# Autodesk Inventor assembly: X Axis
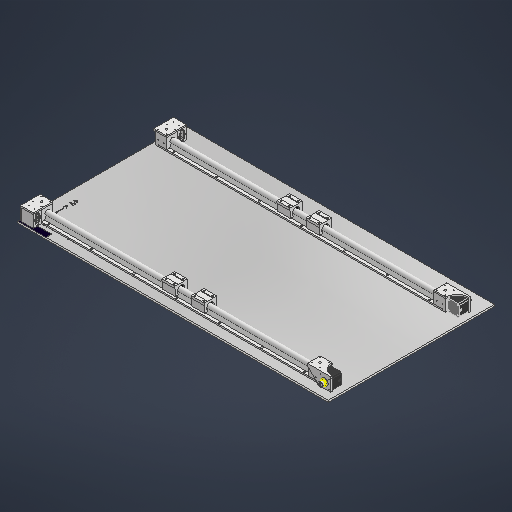
[picture p0: Inventor's stored thumbnail of the model, 512x512]
Saved by Autodesk Inventor 2025.1 (Build 291241000, 241)
## iProperties
Created: 2024-11-25
Part Number: X Axis
Document SubType Name: Assembly
Designer: jerem
Author: jerem
## Documents named in this file (8)
- C:\Users\jerem\Documents\GitHub\Perovskite-Automated-Synthesis-System\CAD\Gantry\X Axis.iam
- C:\Users\jerem\Documents\GitHub\Perovskite-Automated-Synthesis-System\CAD\Non 3D Printed Parts\Base Plate.ipt
- C:\Users\jerem\Documents\GitHub\Perovskite-Automated-Synthesis-System\CAD\Non 3D Printed Parts\Linear Rails\Linear Rail.ipt
- C:\Users\jerem\Documents\GitHub\Perovskite-Automated-Synthesis-System\CAD\Non 3D Printed Parts\Linear Rails\Linear Rail Slider Block.ipt
- C:\Users\jerem\Documents\GitHub\Perovskite-Automated-Synthesis-System\CAD\Gantry\Assembly2 - Copy.iam
- C:\Users\jerem\Documents\GitHub\Perovskite-Automated-Synthesis-System\CAD\Gantry\Belt Tensioner End.iam
- C:\Users\jerem\Documents\GitHub\Perovskite-Automated-Synthesis-System\CAD\Gantry\Assembly2 - Copy_MIR.iam
- C:\Users\jerem\Documents\GitHub\Perovskite-Automated-Synthesis-System\CAD\Gantry\Belt Tensioner End_MIR2.iam
## Components (11 placed, 7 different names)
1. Base Plate:1 — Flush:1, Flush:2, Angle:1, Angle:2, Mate:14, Mate:17, Mate:23, Mate:28
2. Linear Rail:1 — Flush:1, Mate:3, Mate:12, Mate:13, Mate:18, Mate:24, Mate:25, Mate:26
3. Linear Rail:2 — Mate:3, Mate:10, Mate:11, Mate:15, Mate:16, Mate:27, Mate:29
4. Linear Rail Slider Block:1 — Mate:12, Angle:2, Angle:4
5. Linear Rail Slider Block:2 — Mate:13, Angle:4
6. Linear Rail Slider Block:3 — Mate:10, Angle:1, Angle:3
7. Linear Rail Slider Block:4 — Mate:11, Angle:3
8. Assembly2 - Copy:1 [sub-assembly] — Mate:14, Mate:15, Mate:16
9. Belt Tensioner End:1 [sub-assembly] — Mate:17, Mate:18, Flush:2, Mate:26
10. Assembly2 - Copy_MIR:1 [sub-assembly] — Mate:23, Mate:24, Mate:25
11. Belt Tensioner End_MIR2:1 [sub-assembly] — Mate:27, Mate:28, Mate:29
## Relationships (26: Mate 19, Angle 4, Flush 3)
- Flush:1 (20 mm): Base Plate:1 ↔ Linear Rail:1
- Flush:2 (5 mm): Base Plate:1 ↔ Belt Tensioner End:1
- [Mate]: Base Plate:1 ↔ Linear Rail:1
- [Mate]: Base Plate:1 ↔ Linear Rail:2
- [Flush]: Linear Rail:1 ↔ Linear Rail:2
- Mate:3 (400 mm): Linear Rail:1 ↔ Linear Rail:2
- Mate:10: Linear Rail:2 ↔ Linear Rail Slider Block:3
- Mate:11: Linear Rail:2 ↔ Linear Rail Slider Block:4
- Mate:12: Linear Rail:1 ↔ Linear Rail Slider Block:1
- Mate:13: Linear Rail:1 ↔ Linear Rail Slider Block:2
- Angle:1 (0 deg): Base Plate:1 ↔ Linear Rail Slider Block:3
- Angle:2 (0 deg): Base Plate:1 ↔ Linear Rail Slider Block:1
- Angle:3 (0 deg): Linear Rail Slider Block:3 ↔ Linear Rail Slider Block:4
- Angle:4 (0 deg): Linear Rail Slider Block:1 ↔ Linear Rail Slider Block:2
- Mate:14: Base Plate:1 ↔ Assembly2 - Copy:1
- Mate:15: Linear Rail:2 ↔ Assembly2 - Copy:1
- Mate:16: Linear Rail:2 ↔ Assembly2 - Copy:1
- Mate:17: Base Plate:1 ↔ Belt Tensioner End:1
- Mate:18: Linear Rail:1 ↔ Belt Tensioner End:1
- Mate:23: Base Plate:1 ↔ Assembly2 - Copy_MIR:1
- Mate:24: Linear Rail:1 ↔ Assembly2 - Copy_MIR:1
- Mate:25: Linear Rail:1 ↔ Assembly2 - Copy_MIR:1
- Mate:26: Linear Rail:1 ↔ Belt Tensioner End:1
- Mate:27: Linear Rail:2 ↔ Belt Tensioner End_MIR2:1
- Mate:28: Base Plate:1 ↔ Belt Tensioner End_MIR2:1
- Mate:29: Linear Rail:2 ↔ Belt Tensioner End_MIR2:1
